# Autodesk Inventor assembly: Ensamblaje
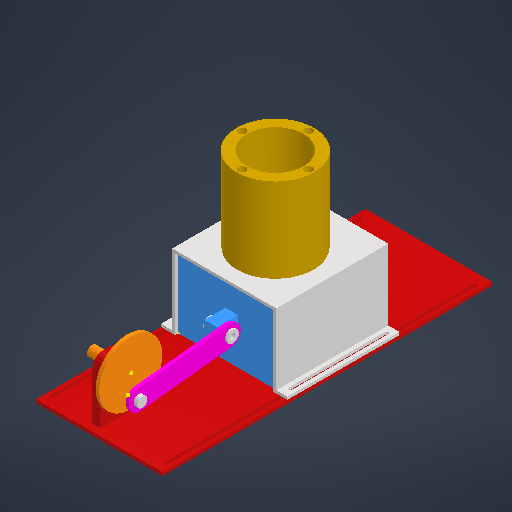
[picture p0: Inventor's stored thumbnail of the model, 512x512]
Saved by Autodesk Inventor 2027.1 (Build 311270010, 270A)
## iProperties
Created: 2026-09-20
Part Number: Ensamblaje
Document SubType Name: Assembly
Designer: dguar
Author: dguar
## Documents named in this file (10)
- C:\Users\tavic\Downloads\2 proyecto\Ensamblaje.iam
- C:\Users\tavic\Downloads\2 proyecto\caja.ipt
- C:\Users\tavic\Downloads\2 proyecto\Part1.ipt
- C:\Users\tavic\Downloads\Balancin.ipt
- C:\Users\tavic\Downloads\2 proyecto\Manivela.ipt
- C:\Users\tavic\Downloads\2 proyecto\Acoplador.ipt
- C:\Users\tavic\Downloads\2 proyecto\cilindro.ipt
- C:\Users\tavic\Downloads\2 proyecto\Tornillo Caja 1.ipt
- C:\Users\tavic\Downloads\2 proyecto\Tornillo Caja 2.ipt
- C:\Users\tavic\Downloads\2 proyecto\Tornillo Manivela.ipt
## Components (9 placed, 9 different names)
1. caja:1 — Rígido:1, Rígido:2
2. Part1:1 — Rígido:1, Corredera:1, De rotación:5
3. Balancin:1 — Corredera:1, De rotación:8
4. Manivela:1 — De rotación:5, De rotación:6, De rotación:7
5. Acoplador:1 — De rotación:3, De rotación:6
6. cilindro:1 — Rígido:2
7. Tornillo Caja 1:1 — De rotación:3, De rotación:4, De rotación:8
8. Tornillo Caja 2:1 — De rotación:4
9. Tornillo Manivela:1 — De rotación:7
## Relationships (9: RevoluteJoint 6, WeldJoint 2, TranslationJoint 1)
- Rígido:1 [WeldJoint] (-131.7625 mm): caja:1 ↔ Part1:1
- Corredera:1 [TranslationJoint]: Part1:1 ↔ Balancin:1
- Rígido:2 [WeldJoint]: caja:1 ↔ cilindro:1
- De rotación:3 [RevoluteJoint]: Acoplador:1 ↔ Tornillo Caja 1:1
- De rotación:4 [RevoluteJoint]: Tornillo Caja 1:1 ↔ Tornillo Caja 2:1
- De rotación:5 [RevoluteJoint]: Part1:1 ↔ Manivela:1
- De rotación:6 [RevoluteJoint]: Manivela:1 ↔ Acoplador:1
- De rotación:7 [RevoluteJoint]: Manivela:1 ↔ Tornillo Manivela:1
- De rotación:8 [RevoluteJoint] (-5 mm): Balancin:1 ↔ Tornillo Caja 1:1
